# Autodesk Inventor assembly: -ZPanel
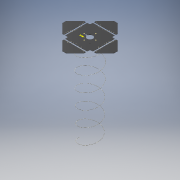
[picture p0: Inventor's stored thumbnail of the model, 180x180]
Saved by Autodesk Inventor 2018 (Build 220112000, 112)
## iProperties
Created: 2018-11-03
Part Number: -ZPanel
Document SubType Name: Assembly
Designer: Bradley
Author: Bradley
## Documents named in this file (14)
- C:\Users\Bradley\Documents\GitHub\CougSat1-Hardware\CougSat1-RadioBoard\CADModel\Native\-ZPanel.iam
- C:\Users\Bradley\Documents\GitHub\CougSat1-Hardware\CougSat1-RadioBoard\CADModel\Native\-ZPanel_PCB.ipt
- C:\Users\Bradley\Documents\GitHub\CougSat1-Hardware\CougSat1-RadioBoard\CADModel\Native\-ZPanel_AntennaDeloyed.ipt
- C:\Users\Bradley\Documents\GitHub\CougSat1-Hardware\CougSat1-RadioBoard\CADModel\Native\-ZPanel_AntennaStored.ipt
- C:\Users\Bradley\Documents\GitHub\Resources\ComponentModels\Connectors\PicoLock-J-4.ipt
- C:\Users\Bradley\Documents\GitHub\Resources\ComponentModels\Connectors\PicoLock-P-4.ipt
- C:\Users\Bradley\Documents\GitHub\Resources\ComponentModels\Connectors\U.FL_Male.ipt
- C:\Users\Bradley\Documents\GitHub\Resources\ComponentModels\Connectors\U.FL_Female.ipt
- C:\Users\Bradley\Documents\GitHub\Resources\ComponentModels\Electronics\Resistor_TH-15mm.ipt
- C:\Users\Bradley\Documents\GitHub\CougSat1-Hardware\CougSat1-RadioBoard\CADModel\Native\-ZPanel_PCBExtender.ipt
- C:\Users\Bradley\Documents\GitHub\CougSat1-Hardware\CougSat1-RadioBoard\CADModel\Native\-ZPanel_SpringLeft.ipt
- C:\Users\Bradley\Documents\GitHub\CougSat1-Hardware\CougSat1-RadioBoard\CADModel\Native\-ZPanel_SpringRight.ipt
- C:\Users\Bradley\Documents\GitHub\CougSat1-Hardware\CougSat1-RadioBoard\CADModel\Native\-ZPanel_SpringDeployed.ipt
- C:\Users\Bradley\Documents\GitHub\Resources\ComponentModels\Electronics\SpringContact_5mm.iam
## Components (53 placed, 13 different names)
1. -ZPanel_PCB:1 — Mate:1, Mate:2, Mate:5, Mate:6, Insert:2, Insert:3, Insert:4, Insert:5, Mate:13, Mate:14, Flush:8, Flush:9, Flush:10, Flush:11, Flush:12, Flush:13, Flush:14, Flush:15, Flush:16, Flush:17, Mate:20, Insert:10, Insert:11, Insert:12, Insert:13
2. -ZPanel_AntennaDeloyed:1 — Mate:11, Mate:12, Mate:1
3. -ZPanel_AntennaStored:1 — Mate:9, Mate:10, Mate:2
4. PicoLock-J-4:1 — Mate:6, Mate:7, Flush:6
5. PicoLock-P-4:1
6. U.FL_Male:1 — Mate:5, Flush:7, Mate:8
7. U.FL_Female:1
8. Resistor_TH-15mm:1 — Insert:4, Insert:5
9. Resistor_TH-15mm:2 — Insert:2, Insert:3
10. SpringContact_5mm:1 [sub-assembly] — Insert:10
11. SpringContact_5mm:2 [sub-assembly] — Insert:11
12. SpringContact_5mm:3 [sub-assembly] — Insert:12
13. SpringContact_5mm:4 [sub-assembly] — Insert:13
14. -ZPanel_PCBExtender:1 — Mate:13, Mate:14, Flush:16
15. -ZPanel_SpringLeft:1 — Flush:8, Mate:15, Flush:9, Insert:6
16. -ZPanel_SpringRight:1 — Flush:12, Flush:13, Mate:17, Insert:9
17. -ZPanel_SpringRight:2 — Mate:18, Flush:14, Flush:15, Insert:8
18. -ZPanel_SpringLeft:2 — Mate:16, Flush:10, Flush:11, Insert:7
19. -ZPanel_PCBExtender:2
20. -ZPanel_SpringLeft:3
21. -ZPanel_SpringRight:3
22. -ZPanel_SpringRight:4
23. -ZPanel_SpringLeft:4
24. -ZPanel_PCBExtender:3
25. -ZPanel_SpringLeft:5
26. -ZPanel_SpringRight:5
27. -ZPanel_SpringRight:6
28. -ZPanel_SpringLeft:6
29. -ZPanel_PCBExtender:4
30. -ZPanel_SpringLeft:7
31. -ZPanel_SpringRight:7
32. -ZPanel_SpringRight:8
33. -ZPanel_SpringLeft:8
34. -ZPanel_SpringDeployed:1 — Insert:6
35. -ZPanel_SpringDeployed:2 — Insert:7
36. -ZPanel_SpringDeployed:3 — Insert:8
37. -ZPanel_SpringDeployed:4 — Insert:9
38. -ZPanel_PCBExtender:5 — Mate:19, Flush:17, Mate:20
39. -ZPanel_SpringDeployed:5
40. -ZPanel_SpringDeployed:6
41. -ZPanel_SpringDeployed:7
42. -ZPanel_SpringDeployed:8
43. -ZPanel_PCBExtender:6
44. -ZPanel_SpringDeployed:9
45. -ZPanel_SpringDeployed:10
46. -ZPanel_SpringDeployed:11
47. -ZPanel_SpringDeployed:12
48. -ZPanel_PCBExtender:7
49. -ZPanel_SpringDeployed:13
50. -ZPanel_SpringDeployed:14
51. -ZPanel_SpringDeployed:15
52. -ZPanel_SpringDeployed:16
53. -ZPanel_PCBExtender:8
## Component patterns: (4 elements, first: -ZPanel_PCBExtender:1 + -ZPanel_SpringLeft:1 + -ZPanel_SpringRight:1 + -ZPanel_SpringRight:2 + -ZPanel_SpringLeft:2), (4 elements, first: -ZPanel_SpringDeployed:1 + -ZPanel_SpringDeployed:2 + -ZPanel_SpringDeployed:3 + -ZPanel_SpringDeployed:4 + -ZPanel_PCBExtender:5)
## Relationships (46: Mate 20, Flush 13, Insert 13)
- Mate:11: -ZPanel_AntennaDeloyed:1
- Mate:12: -ZPanel_AntennaDeloyed:1
- Mate:1 (0.2794 mm): -ZPanel_PCB:1 ↔ -ZPanel_AntennaDeloyed:1
- Mate:9: -ZPanel_AntennaStored:1
- Mate:10: -ZPanel_AntennaStored:1
- Mate:2 (0.2794 mm): -ZPanel_PCB:1 ↔ -ZPanel_AntennaStored:1
- [Flush]: PicoLock-J-4:1 ↔ PicoLock-P-4:1
- [Mate]: PicoLock-J-4:1 ↔ PicoLock-P-4:1
- [Mate] (0.025 mm): PicoLock-J-4:1 ↔ PicoLock-P-4:1
- [Insert] (0.1 mm): U.FL_Male:1 ↔ U.FL_Female:1
- Mate:5: -ZPanel_PCB:1 ↔ U.FL_Male:1
- Mate:6: -ZPanel_PCB:1 ↔ PicoLock-J-4:1
- Mate:7 (-14 mm): PicoLock-J-4:1
- Flush:6 (20 mm): PicoLock-J-4:1
- Flush:7 (15 mm): U.FL_Male:1
- Mate:8 (-22 mm): U.FL_Male:1
- Insert:2 (-1.5 mm): -ZPanel_PCB:1 ↔ Resistor_TH-15mm:2
- Insert:3 (-1.5 mm): -ZPanel_PCB:1 ↔ Resistor_TH-15mm:2
- Insert:4 (-1.5 mm): -ZPanel_PCB:1 ↔ Resistor_TH-15mm:1
- Insert:5 (-1.5 mm): -ZPanel_PCB:1 ↔ Resistor_TH-15mm:1
- Mate:13 (-4 mm): -ZPanel_PCB:1 ↔ -ZPanel_PCBExtender:1
- Mate:14: -ZPanel_PCB:1 ↔ -ZPanel_PCBExtender:1
- Flush:8 (2 mm): -ZPanel_PCB:1 ↔ -ZPanel_SpringLeft:1
- Mate:15 (-24 mm): -ZPanel_SpringLeft:1
- Flush:9: -ZPanel_PCB:1 ↔ -ZPanel_SpringLeft:1
- Mate:16 (-13 mm): -ZPanel_SpringLeft:2
- Flush:10: -ZPanel_PCB:1 ↔ -ZPanel_SpringLeft:2
- Flush:11 (2 mm): -ZPanel_PCB:1 ↔ -ZPanel_SpringLeft:2
- Flush:12: -ZPanel_PCB:1 ↔ -ZPanel_SpringRight:1
- Flush:13 (2 mm): -ZPanel_PCB:1 ↔ -ZPanel_SpringRight:1
- Mate:17 (24 mm): -ZPanel_SpringRight:1
- Mate:18 (13 mm): -ZPanel_SpringRight:2
- Flush:14 (2 mm): -ZPanel_PCB:1 ↔ -ZPanel_SpringRight:2
- Flush:15: -ZPanel_PCB:1 ↔ -ZPanel_SpringRight:2
- Flush:16: -ZPanel_PCB:1 ↔ -ZPanel_PCBExtender:1
- Insert:6: -ZPanel_SpringLeft:1 ↔ -ZPanel_SpringDeployed:1
- Insert:7: -ZPanel_SpringLeft:2 ↔ -ZPanel_SpringDeployed:2
- Insert:8: -ZPanel_SpringRight:2 ↔ -ZPanel_SpringDeployed:3
- Insert:9: -ZPanel_SpringRight:1 ↔ -ZPanel_SpringDeployed:4
- Mate:19: -ZPanel_PCBExtender:5
- Flush:17: -ZPanel_PCB:1 ↔ -ZPanel_PCBExtender:5
- Mate:20 (4.736 mm): -ZPanel_PCB:1 ↔ -ZPanel_PCBExtender:5
- Insert:10: -ZPanel_PCB:1 ↔ SpringContact_5mm:1
- Insert:11: -ZPanel_PCB:1 ↔ SpringContact_5mm:2
- Insert:12: -ZPanel_PCB:1 ↔ SpringContact_5mm:3
- Insert:13: -ZPanel_PCB:1 ↔ SpringContact_5mm:4
## Named parameters: d105_d9 = 0 mm, d106_d10 = 0 mm, d107_d11 = 0.025 mm
